# Autodesk Inventor assembly: MG-Ballsensorplatine
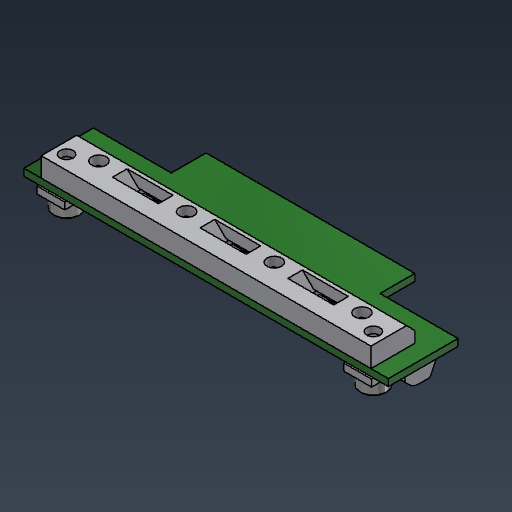
[picture p0: Inventor's stored thumbnail of the model, 512x512]
Saved by Autodesk Inventor 2023.1 (Build 271208000, 208)
## iProperties
Part Number: MG-Ballsensorplatine
Material: Generisch
Document SubType Name: Assembly
Designer: rYan
Mass: 1.72685 g
Surface Area: 31.4704 cm^2
Volume: 1.50793 cm^3
Density: 1.14518 g/cm^3
Author: rYan
## Documents named in this file (7)
- D:\TIGERsGIT\Hardware\mechanik\2024\Inventor\Robot\Electronics\MG-Ballsensorplatine.iam
- D:\TIGERsGIT\Hardware\mechanik\2024\Inventor\Robot\Electronics\Ballsensor IR Platine.ipt
- D:\TIGERsGIT\Hardware\mechanik\2024\Inventor\Robot\Electronics\Ballsensor Platinenwinkel.ipt
- D:\TIGERsGIT\Hardware\mechanik\2024\Inventor\Inhaltscenter\de-DE\ISO 4762(2)\ISO 4762 - M2 x 4ISO.ipt
- D:\TIGERsGIT\Hardware\mechanik\2024\Inventor\Robot\Electronics\Ballsensormaske.ipt
- D:\TIGERsGIT\Hardware\mechanik\2024\Inventor\Purchased Parts\SFH 2701.ipt
- D:\TIGERsGIT\Hardware\mechanik\2024\Inventor\Purchased Parts\SFH 4059.ipt
## Components (13 placed, 6 different names)
1. Ballsensor IR Platine:1 — Fluchtend:1, Fluchtend:2, Fluchtend:3, Passend:4, Passend:5, Passend:6, Passend:7, Einfügen:3, Einfügen:4, Passend:10, Passend:11, Passend:12, Fluchtend:5, Passend:13, Fluchtend:6, Passend:14
2. Ballsensor Platinenwinkel:1 — Passend:4, Passend:6, Winkel:1
3. Ballsensor Platinenwinkel:2 — Passend:5, Passend:7, Winkel:2, Einfügen:5
4. ISO 4762 M2 x 4:3 — Einfügen:3
5. Ballsensormaske:1 — Einfügen:4, Passend:10
6. ISO 4762 M2 x 4:4 — Einfügen:5
7. SFH 4059:1 — Passend:12, Fluchtend:6, Passend:14
8. SFH 4059:2
9. SFH 4059:3
10. SFH 4059:4
11. SFH 2701:1 — Passend:11, Fluchtend:5, Passend:13
12. SFH 2701:2
13. SFH 2701:3
## Component patterns: (4 elements, first: SFH 4059:1), (3 elements, first: SFH 2701:1)
## Relationships (19: Mate 9, Flush 5, Insert 3, Angle 2)
- Fluchtend:1 [Flush]: Ballsensor IR Platine:1
- Fluchtend:2 [Flush]: Ballsensor IR Platine:1
- Fluchtend:3 [Flush]: Ballsensor IR Platine:1
- Passend:4 [Mate]: Ballsensor IR Platine:1 ↔ Ballsensor Platinenwinkel:1
- Passend:5 [Mate]: Ballsensor IR Platine:1 ↔ Ballsensor Platinenwinkel:2
- Passend:6 [Mate]: Ballsensor IR Platine:1 ↔ Ballsensor Platinenwinkel:1
- Passend:7 [Mate]: Ballsensor IR Platine:1 ↔ Ballsensor Platinenwinkel:2
- Winkel:1 [Angle] (0 deg): Ballsensor Platinenwinkel:1
- Winkel:2 [Angle] (0 deg): Ballsensor Platinenwinkel:2
- Einfügen:3 [Insert] (1 mm): Ballsensor IR Platine:1 ↔ ISO 4762 M2 x 4:3
- Einfügen:4 [Insert]: Ballsensor IR Platine:1 ↔ Ballsensormaske:1
- Passend:10 [Mate]: Ballsensor IR Platine:1 ↔ Ballsensormaske:1
- Passend:11 [Mate]: Ballsensor IR Platine:1 ↔ SFH 2701:1
- Passend:12 [Mate]: Ballsensor IR Platine:1 ↔ SFH 4059:1
- Fluchtend:5 [Flush]: Ballsensor IR Platine:1 ↔ SFH 2701:1
- Passend:13 [Mate] (-3.5 mm): Ballsensor IR Platine:1 ↔ SFH 2701:1
- Fluchtend:6 [Flush] (18.9 mm): Ballsensor IR Platine:1 ↔ SFH 4059:1
- Passend:14 [Mate] (-3.5 mm): Ballsensor IR Platine:1 ↔ SFH 4059:1
- Einfügen:5 [Insert]: Ballsensor Platinenwinkel:2 ↔ ISO 4762 M2 x 4:4
